# Autodesk Inventor assembly: Intake Prototypes
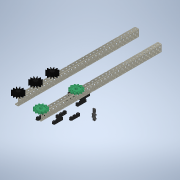
[picture p0: Inventor's stored thumbnail of the model, 180x180]
Saved by Autodesk Inventor 2020 (Build 240168000, 168)
## iProperties
Created: 2019-09-15
Part Number: Intake Prototypes
Document SubType Name: Assembly
Designer: Corey
Author: Corey
## Documents named in this file (6)
- D:\Robotics\CAD\Intake Prototypes.iam
- D:\Robotics\CAD\Parts\Structure\C-Channels\Aluminum\2-Wide\Aluminum C-Channel 1x2x1x35.ipt
- D:\Robotics\CAD\Parts\Motion\Wheels & Rollers\Intake Roller.ipt
- D:\Robotics\CAD\Parts\Motion\Sprockets\High Strength 12-tooth Sprocket.ipt
- D:\Robotics\CAD\Parts\Motion\Chain & Tank Tread\Tank Tread Traction Link.ipt
- D:\Robotics\CAD\Parts\Motion\Bearing Flat.ipt
## Components (16 placed, 5 different names)
1. Aluminum C-Channel 1x2x1x35:1
2. Intake Roller:1
3. Intake Roller:2
4. Intake Roller:3
5. Aluminum C-Channel 1x2x1x35:2 — Mate:1
6. High Strength 12-tooth Sprocket:1
7. High Strength 12-tooth Sprocket:2
8. Tank Tread Traction Link:1
9. Bearing Flat:1 — Mate:1
10. Bearing Flat:2
11. Bearing Flat:3
12. Bearing Flat:4
13. Bearing Flat:5
14. Bearing Flat:6
15. Bearing Flat:7
16. Bearing Flat:8
## Relationships (1: Mate 1)
- Mate:1: Aluminum C-Channel 1x2x1x35:2 ↔ Bearing Flat:1
